# Autodesk Inventor assembly: BBM Assembly v1p1
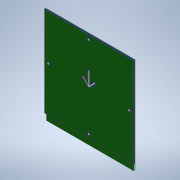
[picture p0: Inventor's stored thumbnail of the model, 180x180]
Saved by Autodesk Inventor 2022 (Build 260153000, 153)
## iProperties
Created: 2022-05-17
Part Number: BBM Assembly v1p1
Document SubType Name: Assembly
Designer: Caleb
Author: Caleb
## iProperties of the stored document pads_area003#F.Cu#3#REF__.ipt
Created: 2022-05-17
Part Number: pads_area003#F.Cu#3#REF__
Material: Generic
Document SubType Name: Modeling
Designer: Caleb
Density: 1 g/cm^3
Appearance: Default
Author: Caleb
## iProperties of the stored document copper_combo#F.Cu.ipt
Created: 2022-05-17
Part Number: copper_combo#F.Cu
Material: Generic
Document SubType Name: Modeling
Designer: Caleb
Density: 1 g/cm^3
Appearance: Default
Author: Caleb
## iProperties of the stored document etl_etroc_mockup_v1p1.iam
Created: 2022-05-17
Part Number: etl_etroc_mockup_v1p1
Description: FreeCAD Model
Document SubType Name: Assembly
Designer: Caleb
Authority: Unknown
Title: Open CASCADE Shape Model
Author: Author
Sending System: FreeCAD
Preprocessor: Open CASCADE STEP processor 7.5
## iProperties of the stored document pads_wire002#F.Cu#2#REF__.ipt
Created: 2022-05-17
Part Number: pads_wire002#F.Cu#2#REF__
Material: Generic
Document SubType Name: Modeling
Designer: Caleb
Density: 1 g/cm^3
Appearance: Default
Author: Caleb
## iProperties of the stored document zone_wire#F.Cu#__.ipt
Created: 2022-05-17
Part Number: zone_wire#F.Cu#__
Material: Generic
Document SubType Name: Modeling
Designer: Caleb
Density: 1 g/cm^3
Appearance: Default
Author: Caleb
## iProperties of the stored document zones_solid#F.Cu.ipt
Created: 2022-05-17
Part Number: zones_solid#F.Cu
Material: Generic
Document SubType Name: Modeling
Designer: Caleb
Density: 1 g/cm^3
Appearance: Default
Author: Caleb
## iProperties of the stored document zone_area#F.Cu#__.ipt
Created: 2022-05-17
Part Number: zone_area#F.Cu#__
Material: Generic
Document SubType Name: Modeling
Designer: Caleb
Density: 1 g/cm^3
Appearance: Default
Author: Caleb
## iProperties of the stored document pads_wire001#F.Cu#1#REF__.ipt
Created: 2022-05-17
Part Number: pads_wire001#F.Cu#1#REF__
Material: Generic
Document SubType Name: Modeling
Designer: Caleb
Density: 1 g/cm^3
Appearance: Default
Author: Caleb
## iProperties of the stored document board_solid.ipt
Created: 2022-05-17
Part Number: board_solid
Material: Generic
Document SubType Name: Modeling
Designer: Caleb
Density: 1 g/cm^3
Appearance: Default
Author: Caleb
## iProperties of the stored document pads_wire003#F.Cu#3#REF__.ipt
Created: 2022-05-17
Part Number: pads_wire003#F.Cu#3#REF__
Material: Generic
Document SubType Name: Modeling
Designer: Caleb
Density: 1 g/cm^3
Appearance: Default
Author: Caleb
## iProperties of the stored document pads_wire#F.Cu#0#REF__.ipt
Created: 2022-05-17
Part Number: pads_wire#F.Cu#0#REF__
Material: Generic
Document SubType Name: Modeling
Designer: Caleb
Density: 1 g/cm^3
Appearance: Default
Author: Caleb
## iProperties of the stored document pads_area001#F.Cu#1#REF__.ipt
Created: 2022-05-17
Part Number: pads_area001#F.Cu#1#REF__
Material: Generic
Document SubType Name: Modeling
Designer: Caleb
Density: 1 g/cm^3
Appearance: Default
Author: Caleb
## iProperties of the stored document pads_area#F.Cu#0#REF__.ipt
Created: 2022-05-17
Part Number: pads_area#F.Cu#0#REF__
Material: Generic
Document SubType Name: Modeling
Designer: Caleb
Density: 1 g/cm^3
Appearance: Default
Author: Caleb
## iProperties of the stored document pads_solid#F.Cu.ipt
Created: 2022-05-17
Part Number: pads_solid#F.Cu
Material: Generic
Document SubType Name: Modeling
Designer: Caleb
Density: 1 g/cm^3
Appearance: Default
Author: Caleb
## iProperties of the stored document board_wire#outline.ipt
Created: 2022-05-17
Part Number: board_wire#outline
Material: Generic
Document SubType Name: Modeling
Designer: Caleb
Density: 1 g/cm^3
Appearance: Default
Author: Caleb
## iProperties of the stored document pads_area002#F.Cu#2#REF__.ipt
Created: 2022-05-17
Part Number: pads_area002#F.Cu#2#REF__
Material: Generic
Document SubType Name: Modeling
Designer: Caleb
Density: 1 g/cm^3
Appearance: Default
Author: Caleb
## iProperties of the stored document pcb_combo.ipt
Created: 2022-05-17
Part Number: pcb_combo
Material: Generic
Document SubType Name: Modeling
Designer: Caleb
Density: 1 g/cm^3
Appearance: Default
Author: Caleb
## iProperties of the stored document pads_area004#F.Cu.ipt
Created: 2022-05-17
Part Number: pads_area004#F.Cu
Material: Generic
Document SubType Name: Modeling
Designer: Caleb
Density: 1 g/cm^3
Appearance: Default
Author: Caleb
## iProperties of the stored document board_area.ipt
Created: 2022-05-17
Part Number: board_area
Material: Generic
Document SubType Name: Modeling
Designer: Caleb
Density: 1 g/cm^3
Appearance: Default
Author: Caleb
## iProperties of the stored document etl_lgad_mockup_v1p1.ipt
Created: 2022-05-17
Part Number: etl_lgad_mockup_v1p1
Material: Generic
Description: FreeCAD Model
Document SubType Name: Modeling
Designer: Caleb
Authority: Unknown
Density: 1 g/cm^3
Appearance: Default
Title: Open CASCADE Shape Model
Author: Author
Sending System: FreeCAD
Preprocessor: Open CASCADE STEP processor 7.5
## Documents named in this file (23)
- **C:\Users\Caleb\Desktop\nebraska-silicon-lab\Hardware\ETL\modules\throughput mockups\BBM Assembly v1p1.iam*LocalDocs*xAaaaaeaaAaaaaaaaAaaaacsjGa*pads_area003#F.Cu#3#REF__.ipt
- **C:\Users\Caleb\Desktop\nebraska-silicon-lab\Hardware\ETL\modules\throughput mockups\BBM Assembly v1p1.iam*LocalDocs*xAaaaacdaAaaaaaaaAaaaq1cyTa*copper_combo#F.Cu.ipt
- **C:\Users\Caleb\Desktop\nebraska-silicon-lab\Hardware\ETL\modules\throughput mockups\BBM Assembly v1p1.iam*LocalDocs*xAaaaa3aaAaaaaaaaAaaaqdqrNh*etl_etroc_mockup_v1p1.iam
- **C:\Users\Caleb\Desktop\nebraska-silicon-lab\Hardware\ETL\modules\throughput mockups\BBM Assembly v1p1.iam*LocalDocs*xAaaaq3caAaaaaaaaAaaaaqbgBg*board_wire#outline.ipt
- **C:\Users\Caleb\Desktop\nebraska-silicon-lab\Hardware\ETL\modules\throughput mockups\BBM Assembly v1p1.iam*LocalDocs*xAaaaqfcaAaaaaaaaAaaaqjmdOe*pads_area#F.Cu#0#REF__.ipt
- **C:\Users\Caleb\Desktop\nebraska-silicon-lab\Hardware\ETL\modules\throughput mockups\BBM Assembly v1p1.iam*LocalDocs*xAaaaazcaAaaaaaaaAaaaaw25Wh*pads_area001#F.Cu#1#REF__.ipt
- **C:\Users\Caleb\Desktop\nebraska-silicon-lab\Hardware\ETL\modules\throughput mockups\BBM Assembly v1p1.iam*LocalDocs*xAaaaqjbaAaaaaaaaAaaaahso4h*pads_area002#F.Cu#2#REF__.ipt
- **C:\Users\Caleb\Desktop\nebraska-silicon-lab\Hardware\ETL\modules\throughput mockups\BBM Assembly v1p1.iam*LocalDocs*xAaaaqncaAaaaaaaaAaaaqcysRd*pads_area004#F.Cu.ipt
- **C:\Users\Caleb\Desktop\nebraska-silicon-lab\Hardware\ETL\modules\throughput mockups\BBM Assembly v1p1.iam*LocalDocs*xAaaaadbaAaaaaaaaAaaaqoaqYf*zone_area#F.Cu#__.ipt
- **C:\Users\Caleb\Desktop\nebraska-silicon-lab\Hardware\ETL\modules\throughput mockups\BBM Assembly v1p1.iam*LocalDocs*xAaaaatdaAaaaaaaaAaaaqynp2g*pads_wire#F.Cu#0#REF__.ipt
- **C:\Users\Caleb\Desktop\nebraska-silicon-lab\Hardware\ETL\modules\throughput mockups\BBM Assembly v1p1.iam*LocalDocs*xAaaaqcaaAaaaaaaaAaaaagpzXb*pads_solid#F.Cu.ipt
- **C:\Users\Caleb\Desktop\nebraska-silicon-lab\Hardware\ETL\modules\throughput mockups\BBM Assembly v1p1.iam*LocalDocs*xAaaaavdaAaaaaaaaAaaaq45yEb*pads_wire003#F.Cu#3#REF__.ipt
- **C:\Users\Caleb\Desktop\nebraska-silicon-lab\Hardware\ETL\modules\throughput mockups\BBM Assembly v1p1.iam*LocalDocs*xAaaaqwdaAaaaaaaaAaaaa5nfOc*board_area.ipt
- **C:\Users\Caleb\Desktop\nebraska-silicon-lab\Hardware\ETL\modules\throughput mockups\BBM Assembly v1p1.iam*LocalDocs*xAaaaq2daAaaaaaaaAaaaqb5oAc*board_solid.ipt
- **C:\Users\Caleb\Desktop\nebraska-silicon-lab\Hardware\ETL\modules\throughput mockups\BBM Assembly v1p1.iam*LocalDocs*xAaaaqlcaAaaaaaaaAaaaqss2Ud*pads_wire001#F.Cu#1#REF__.ipt
- **C:\Users\Caleb\Desktop\nebraska-silicon-lab\Hardware\ETL\modules\throughput mockups\BBM Assembly v1p1.iam*LocalDocs*xAaaaa1caAaaaaaaaAaaaqfv52g*pads_wire002#F.Cu#2#REF__.ipt
- **C:\Users\Caleb\Desktop\nebraska-silicon-lab\Hardware\ETL\modules\throughput mockups\BBM Assembly v1p1.iam*LocalDocs*xAaaaabaaAaaaaaaaAaaaa1f3Ce*zone_wire#F.Cu#__.ipt
- **C:\Users\Caleb\Desktop\nebraska-silicon-lab\Hardware\ETL\modules\throughput mockups\BBM Assembly v1p1.iam*LocalDocs*xAaaaadcaAaaaaaaaAaaaa3vzOb*zones_solid#F.Cu.ipt
- **C:\Users\Caleb\Desktop\nebraska-silicon-lab\Hardware\ETL\modules\throughput mockups\BBM Assembly v1p1.iam*LocalDocs*xAaaaqrdaAaaaaaaaAaaaq1cc4b*pcb_combo.ipt
- **C:\Users\Caleb\Desktop\nebraska-silicon-lab\Hardware\ETL\modules\throughput mockups\BBM Assembly v1p1.iam*LocalDocs*xAaaaqrdaAaaaaaaaAaaaq1cc5b*etl_lgad_mockup_v1p1.ipt
- C:\Users\Caleb\Desktop\nebraska-silicon-lab\Hardware\ETL\modules\throughput mockups\BBM Assembly v1p1.iam
- C:\Users\Caleb\Desktop\nebraska-silicon-lab\Hardware\ETL\modules\throughput mockups\etl_etroc_mockup_v1p1.step
- C:\Users\Caleb\Desktop\nebraska-silicon-lab\Hardware\ETL\modules\throughput mockups\etl_lgad_mockup_v1p1.step
## Components (2 placed, 2 different names)
1. etl_etroc_mockup_v1p1:1 [sub-assembly] — Mate:1, Angle:1, Flush:1, Flush:2
2. etl_lgad_mockup_v1p1:1 — Mate:1, Angle:1, Flush:1, Flush:2
## Relationships (4: Flush 2, Mate 1, Angle 1)
- Mate:1: etl_etroc_mockup_v1p1:1 ↔ etl_lgad_mockup_v1p1:1
- Angle:1 (0 deg): etl_etroc_mockup_v1p1:1 ↔ etl_lgad_mockup_v1p1:1
- Flush:1 (-0.2 mm): etl_etroc_mockup_v1p1:1 ↔ etl_lgad_mockup_v1p1:1
- Flush:2 (0.2 mm): etl_etroc_mockup_v1p1:1 ↔ etl_lgad_mockup_v1p1:1
